# Autodesk Inventor assembly: Drive Outside Bracket
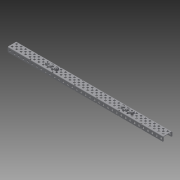
[picture p0: Inventor's stored thumbnail of the model, 180x180]
Saved by Autodesk Inventor 2015 (Build 190159000, 159)
## iProperties
Created: 2016-09-22
Part Number: Drive Outside Bracket
Document SubType Name: Assembly
Designer: Leo
Author: Leo
## Documents named in this file (5)
- C:\Users\Leo\Google Drive\StarStuckProject\Starstruck\Prototypes\Drive Outside Bracket.iam
- C:\Users\Leo\Google Drive\StarStuckProject\Starstruck\Imported Components\C-Channel 1x2x1x35\C-Channel 1x2x1x35.ipt
- C:\Users\Leo\Google Drive\StarStuckProject\Starstruck\Imported Components\Flat Bearing\Flat Bearing.ipt
- C:\Users\Leo\Google Drive\StarStuckProject\Starstruck\Imported Components\Large Screw .750In\Large Screw .750In.ipt
- C:\Users\Leo\Google Drive\StarStuckProject\Starstruck\Imported Components\Regular Nut\Regular Nut.ipt
## Components (11 placed, 4 different names)
1. C-Channel 1x2x1x35:1 — Mate:1, Mate:2, Tangent:1, Tangent:2, Tangent:3, Tangent:4, Tangent:5, Tangent:6, Tangent:7, Tangent:8, Mate:3, Mate:4, Mate:5, Mate:6
2. Flat Bearing:1 — Mate:1, Insert:4, Insert:1
3. Flat Bearing:2 — Mate:2, Insert:2, Insert:3
4. Large Screw .750In:1 — Insert:2, Tangent:5, Tangent:6, Tangent:10
5. Large Screw .750In:2 — Insert:3, Tangent:7, Tangent:8, Tangent:9
6. Large Screw .750In:3 — Insert:1, Tangent:1, Tangent:2, Tangent:11
7. Large Screw .750In:4 — Insert:4, Tangent:3, Tangent:4, Tangent:12
8. Regular Nut:1 — Mate:3, Tangent:9
9. Regular Nut:2 — Mate:4, Tangent:10
10. Regular Nut:3 — Mate:5, Tangent:11
11. Regular Nut:4 — Mate:6, Tangent:12
## Relationships (22: Tangent 12, Mate 6, Insert 4)
- Mate:1: C-Channel 1x2x1x35:1 ↔ Flat Bearing:1
- Mate:2: C-Channel 1x2x1x35:1 ↔ Flat Bearing:2
- Insert:4: Flat Bearing:1 ↔ Large Screw .750In:4
- Insert:1: Flat Bearing:1 ↔ Large Screw .750In:3
- Insert:2: Flat Bearing:2 ↔ Large Screw .750In:1
- Insert:3: Flat Bearing:2 ↔ Large Screw .750In:2
- Tangent:1: C-Channel 1x2x1x35:1 ↔ Large Screw .750In:3
- Tangent:2: C-Channel 1x2x1x35:1 ↔ Large Screw .750In:3
- Tangent:3: C-Channel 1x2x1x35:1 ↔ Large Screw .750In:4
- Tangent:4: C-Channel 1x2x1x35:1 ↔ Large Screw .750In:4
- Tangent:5: C-Channel 1x2x1x35:1 ↔ Large Screw .750In:1
- Tangent:6: C-Channel 1x2x1x35:1 ↔ Large Screw .750In:1
- Tangent:7: C-Channel 1x2x1x35:1 ↔ Large Screw .750In:2
- Tangent:8: C-Channel 1x2x1x35:1 ↔ Large Screw .750In:2
- Mate:3: C-Channel 1x2x1x35:1 ↔ Regular Nut:1
- Mate:4: C-Channel 1x2x1x35:1 ↔ Regular Nut:2
- Mate:5: C-Channel 1x2x1x35:1 ↔ Regular Nut:3
- Mate:6: C-Channel 1x2x1x35:1 ↔ Regular Nut:4
- Tangent:9: Large Screw .750In:2 ↔ Regular Nut:1
- Tangent:10: Large Screw .750In:1 ↔ Regular Nut:2
- Tangent:11: Large Screw .750In:3 ↔ Regular Nut:3
- Tangent:12: Large Screw .750In:4 ↔ Regular Nut:4
